# Autodesk Inventor assembly: completeAssembly_StraightBody
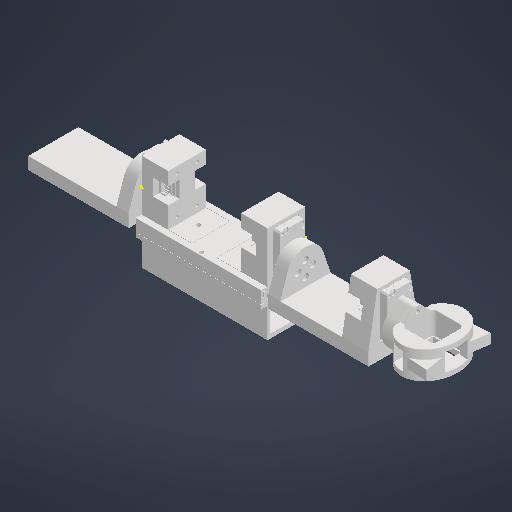
[picture p0: Inventor's stored thumbnail of the model, 512x512]
Saved by Autodesk Inventor 2026 (Build 300175000, 175)
## iProperties
Created: 2025-04-15
Part Number: completeAssembly_StraightBody
Document SubType Name: Assembly
Designer: Elizabeth
Author: Elizabeth
## Documents named in this file (10)
- C:\Users\Elizabeth\FrontierLab\firstMockup\completeAssembly_StraightBody.iam
- C:\Users\Elizabeth\FrontierLab\firstMockup\centralBody.ipt
- C:\Users\Elizabeth\FrontierLab\firstMockup\controllerHousing.ipt
- C:\Users\Elizabeth\FrontierLab\firstMockup\DYNAMIXEL\DYNAMIXEL_XL330XL,XC-330.iam
- C:\Users\Elizabeth\FrontierLab\firstMockup\rearTorso.ipt
- C:\Users\Elizabeth\FrontierLab\firstMockup\frontTorso.ipt
- C:\Users\Elizabeth\FrontierLab\firstMockup\neck.ipt
- C:\Users\Elizabeth\FrontierLab\firstMockup\head.ipt
- C:\Users\Elizabeth\FrontierLab\firstMockup\motorHousingStraight.ipt
- C:\Users\Elizabeth\FrontierLab\firstMockup\extBoardHousing .ipt
## Components (12 placed, 9 different names)
1. centralBody:1 — Mate:5, Flush:3, Flush:4, Flush:6, Flush:7, Flush:8, Mate:27, Flush:9, Flush:10, Mate:28, Flush:11, Mate:38, Mate:39, Mate:40
2. controllerHousing:1 — Mate:5, Flush:3, Flush:4
3. DYNAMIXEL_XL330XL,XC-330:1 [sub-assembly] — Mate:16, Mate:32, Mate:33, Mate:34, Mate:37
4. DYNAMIXEL_XL330XL,XC-330:2 [sub-assembly] — Mate:29, Mate:30, Mate:31, Mate:35, Mate:36
5. frontTorso:1 — Mate:16, Flush:6, Mate:17, Mate:18, Mate:19, Mate:37
6. DYNAMIXEL_XL330XL,XC-330:3 [sub-assembly] — Mate:17, Mate:18, Mate:19, Mate:22, Mate:24
7. neck:1 — Mate:22, Mate:23, Mate:24, Mate:25, Mate:26
8. head:1 — Mate:23, Mate:25, Mate:26
9. motorHousingStraight:1 — Flush:7, Flush:8, Mate:27, Mate:29, Mate:30, Mate:31
10. motorHousingStraight:2 — Flush:9, Flush:10, Mate:28, Mate:32, Mate:33, Mate:34
11. rearTorso:1 — Mate:35, Flush:11, Mate:36
12. extBoardHousing :1 — Mate:38, Mate:39, Mate:40
## Relationships (32: Mate 24, Flush 8)
- Mate:5: centralBody:1 ↔ controllerHousing:1
- Flush:3: centralBody:1 ↔ controllerHousing:1
- Flush:4: centralBody:1 ↔ controllerHousing:1
- Mate:16 (0.3 mm): DYNAMIXEL_XL330XL,XC-330:1 ↔ frontTorso:1
- Flush:6: centralBody:1 ↔ frontTorso:1
- Mate:17 (0.1 mm): frontTorso:1 ↔ DYNAMIXEL_XL330XL,XC-330:3
- Mate:18 (0.1 mm): frontTorso:1 ↔ DYNAMIXEL_XL330XL,XC-330:3
- Mate:19 (0.1 mm): frontTorso:1 ↔ DYNAMIXEL_XL330XL,XC-330:3
- Mate:22 (0.3 mm): DYNAMIXEL_XL330XL,XC-330:3 ↔ neck:1
- Mate:23: neck:1 ↔ head:1
- Mate:24: DYNAMIXEL_XL330XL,XC-330:3 ↔ neck:1
- Mate:25: neck:1 ↔ head:1
- Mate:26: neck:1 ↔ head:1
- Flush:7: centralBody:1 ↔ motorHousingStraight:1
- Flush:8: centralBody:1 ↔ motorHousingStraight:1
- Mate:27 (0.3 mm): centralBody:1 ↔ motorHousingStraight:1
- Flush:9: centralBody:1 ↔ motorHousingStraight:2
- Flush:10: centralBody:1 ↔ motorHousingStraight:2
- Mate:28 (0.3 mm): centralBody:1 ↔ motorHousingStraight:2
- Mate:29 (0.1 mm): DYNAMIXEL_XL330XL,XC-330:2 ↔ motorHousingStraight:1
- Mate:30 (0.1 mm): DYNAMIXEL_XL330XL,XC-330:2 ↔ motorHousingStraight:1
- Mate:31 (0.2 mm): DYNAMIXEL_XL330XL,XC-330:2 ↔ motorHousingStraight:1
- Mate:32 (0.1 mm): DYNAMIXEL_XL330XL,XC-330:1 ↔ motorHousingStraight:2
- Mate:33 (0.1 mm): DYNAMIXEL_XL330XL,XC-330:1 ↔ motorHousingStraight:2
- Mate:34 (0.2 mm): DYNAMIXEL_XL330XL,XC-330:1 ↔ motorHousingStraight:2
- Mate:35 (0.3 mm): DYNAMIXEL_XL330XL,XC-330:2 ↔ rearTorso:1
- Flush:11: centralBody:1 ↔ rearTorso:1
- Mate:36: DYNAMIXEL_XL330XL,XC-330:2 ↔ rearTorso:1
- Mate:37: DYNAMIXEL_XL330XL,XC-330:1 ↔ frontTorso:1
- Mate:38: centralBody:1 ↔ extBoardHousing :1
- Mate:39: centralBody:1 ↔ extBoardHousing :1
- Mate:40: centralBody:1 ↔ extBoardHousing :1
